# Autodesk Inventor assembly: poleStandHorizAssyB
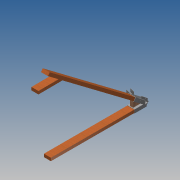
[picture p0: Inventor's stored thumbnail of the model, 180x180]
Saved by Autodesk Inventor 2014 SP1 (Build 180222100, 222)
## iProperties
Created: 2014-08-25
Part Number: poleStandHorizAssyB
Document SubType Name: Assembly
Designer: Dave
Author: Dave
## Documents named in this file (5)
- C:\Users\Dave\Desktop\hera-cad\support\poleStandHorizAssy.iam
- C:\Users\Dave\Desktop\hera-cad\support\poleStandHoriz2.ipt
- C:\Users\Dave\Desktop\hera-cad\support\endAssembly.iam
- C:\Users\Dave\Desktop\hera-cad\support\poleStand37.ipt
- C:\Users\Dave\Desktop\hera-cad\support\poleStandHoriz3.ipt
## Components (4 placed, 4 different names)
1. poleStandHoriz2:1 — Mate:1, Mate:2, Mate:3
2. endAssembly:1 [sub-assembly] — Mate:1, Mate:2, Mate:3, Mate:4, Mate:5, Mate:6
3. poleStand37:1 — Mate:4, Mate:5, Mate:6, Mate:7, Flush:1
4. poleStandHoriz3:1 — Mate:7, Flush:1
## Relationships (8: Mate 7, Flush 1)
- Mate:1: poleStandHoriz2:1 ↔ endAssembly:1
- Mate:2: poleStandHoriz2:1 ↔ endAssembly:1
- Mate:3: poleStandHoriz2:1 ↔ endAssembly:1
- Mate:4: endAssembly:1 ↔ poleStand37:1
- Mate:5: endAssembly:1 ↔ poleStand37:1
- Mate:6: endAssembly:1 ↔ poleStand37:1
- Mate:7: poleStand37:1 ↔ poleStandHoriz3:1
- Flush:1: poleStand37:1 ↔ poleStandHoriz3:1
